# Autodesk Inventor assembly: Assembly1
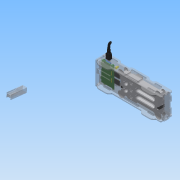
[picture p0: Inventor's stored thumbnail of the model, 180x180]
Saved by Autodesk Inventor 2016 (Build 200138000, 138)
## iProperties
Created: 2015-06-16
Part Number: Assembly1
Document SubType Name: Assembly
Designer: Openlab
Author: Openlab
## Documents named in this file (13)
- D:\Alexey\HS-Spectrophotometer\parts\Paris\Assembly.iam
- D:\Alexey\HS-Spectrophotometer\parts\Paris\LED_board.ipt
- D:\Alexey\HS-Spectrophotometer\parts\Paris\Sensor_board.ipt
- D:\Alexey\HS-Spectrophotometer\parts\Paris\Box_top.ipt
- D:\Alexey\HS-Spectrophotometer\parts\Paris\Box_bottom.ipt
- D:\Alexey\HS-Spectrophotometer\parts\Paris\Box_left_wall.ipt
- D:\Alexey\HS-Spectrophotometer\parts\Paris\Box_right_wall.ipt
- D:\Alexey\HS-Spectrophotometer\parts\Paris\Microcontroller_board_Paris.iam
- D:\Alexey\HS-Spectrophotometer\parts\Paris\Box_back_wall.ipt
- D:\Alexey\HS-Spectrophotometer\parts\Paris\Box_front_wall.ipt
- D:\Alexey\HS-Spectrophotometer\parts\Common\Cuvette.ipt
- D:\Alexey\HS-Spectrophotometer\parts\Paris\Core_bottom-im.ipt
- D:\Alexey\HS-Spectrophotometer\parts\Paris\Core_top-im.ipt
## Components (13 placed, 12 different names)
1. LED_board:1 — Mate:95, Mate:96, Mate:97
2. Sensor_board:1 — Mate:98, Mate:99, Mate:100
3. Box_top:1 — Mate:72, Mate:76, Mate:77, Mate:78, Mate:84, Mate:86, Mate:92
4. Box_bottom:1 — Mate:79, Mate:80, Mate:81, Mate:102, Mate:103
5. Box_left_wall:1 — Mate:83, Mate:84, Mate:85, Mate:91
6. Box_right_wall:1 — Mate:72
7. Microcontroller_board_Paris:1 [sub-assembly] — Mate:89, Mate:90, Mate:91
8. Box_back_wall:1 — Mate:76, Mate:77, Mate:78, Mate:79, Mate:80, Mate:81, Mate:83, Mate:85, Mate:87, Mate:88, Angle:1
9. Box_front_wall:1 — Mate:92, Mate:93, Mate:94
10. Box_left_wall:2 — Mate:86, Mate:87, Mate:88, Mate:89, Mate:90, Mate:93, Mate:94
11. Cuvette:1
12. Core_bottom-im:1 — Mate:95, Mate:96, Mate:97, Mate:98, Mate:99, Mate:100, Mate:101, Flush:1, Flush:2, Mate:102, Mate:103, Angle:1
13. Core_top-im:1 — Mate:101, Flush:1, Flush:2
## Relationships (31: Mate 28, Flush 2, Angle 1)
- Mate:72: Box_top:1 ↔ Box_right_wall:1
- Mate:76: Box_top:1 ↔ Box_back_wall:1
- Mate:77: Box_top:1 ↔ Box_back_wall:1
- Mate:78: Box_top:1 ↔ Box_back_wall:1
- Mate:79: Box_bottom:1 ↔ Box_back_wall:1
- Mate:80: Box_bottom:1 ↔ Box_back_wall:1
- Mate:81: Box_bottom:1 ↔ Box_back_wall:1
- Mate:83: Box_left_wall:1 ↔ Box_back_wall:1
- Mate:84: Box_top:1 ↔ Box_left_wall:1
- Mate:85: Box_left_wall:1 ↔ Box_back_wall:1
- Mate:86: Box_top:1 ↔ Box_left_wall:2
- Mate:87: Box_back_wall:1 ↔ Box_left_wall:2
- Mate:88: Box_back_wall:1 ↔ Box_left_wall:2
- Mate:89: Microcontroller_board_Paris:1 ↔ Box_left_wall:2
- Mate:90: Microcontroller_board_Paris:1 ↔ Box_left_wall:2
- Mate:91: Box_left_wall:1 ↔ Microcontroller_board_Paris:1
- Mate:92: Box_top:1 ↔ Box_front_wall:1
- Mate:93: Box_front_wall:1 ↔ Box_left_wall:2
- Mate:94: Box_front_wall:1 ↔ Box_left_wall:2
- Mate:95: LED_board:1 ↔ Core_bottom-im:1
- Mate:96 (0.5 mm): LED_board:1 ↔ Core_bottom-im:1
- Mate:97: LED_board:1 ↔ Core_bottom-im:1
- Mate:98: Sensor_board:1 ↔ Core_bottom-im:1
- Mate:99 (0.5 mm): Sensor_board:1 ↔ Core_bottom-im:1
- Mate:100: Sensor_board:1 ↔ Core_bottom-im:1
- Mate:101: Core_bottom-im:1 ↔ Core_top-im:1
- Flush:1: Core_bottom-im:1 ↔ Core_top-im:1
- Flush:2: Core_bottom-im:1 ↔ Core_top-im:1
- Mate:102: Box_bottom:1 ↔ Core_bottom-im:1
- Mate:103: Box_bottom:1 ↔ Core_bottom-im:1
- Angle:1 (180 deg): Box_back_wall:1 ↔ Core_bottom-im:1
